# Autodesk Inventor assembly: camera assemble v2
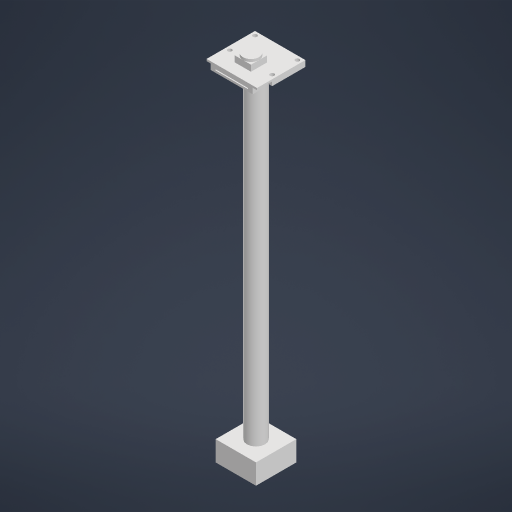
[picture p0: Inventor's stored thumbnail of the model, 512x512]
Saved by Autodesk Inventor 2024 (Build 280153000, 153)
## iProperties
Created: 2023-06-18
Part Number: camera assemble v2
Document SubType Name: Assembly
Designer: 6gioc
Author: 6gioc
## Documents named in this file (3)
- C:\Users\6gioc\OneDrive\AAST\PART\camera assemble v2.iam
- C:\Users\6gioc\OneDrive\AAST\PART\r_camera v2.ipt
- C:\Users\6gioc\OneDrive\AAST\PART\camera arm v1.ipt
## Components (2 placed, 2 different names)
1. r_camera v2:1 — 삽입:1, 삽입:2
2. camera arm v1:1 — 삽입:1, 삽입:2
## Relationships (2: Insert 2)
- 삽입:1 [Insert]: r_camera v2:1 ↔ camera arm v1:1
- 삽입:2 [Insert]: r_camera v2:1 ↔ camera arm v1:1
